# Autodesk Inventor assembly: Montage final
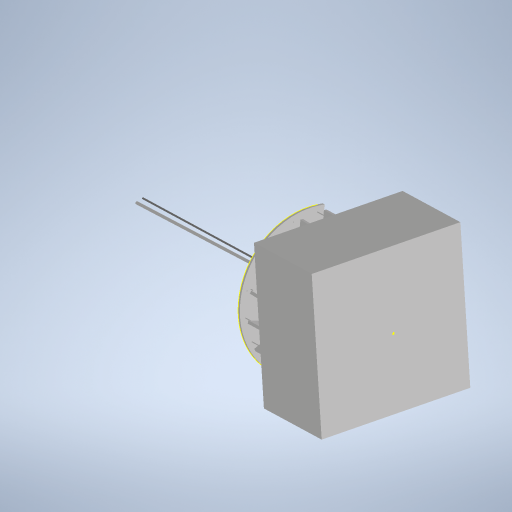
[picture p0: Inventor's stored thumbnail of the model, 512x512]
Saved by Autodesk Inventor 2023 (Build 270158000, 158)
## iProperties
Created: 2022-11-02
Part Number: Montage final
Document SubType Name: Assembly
Designer: Julia
Author: Julia
## Documents named in this file (7)
- C:\Users\Julia\OneDrive\Bureau\PIE\Montage final.iam
- C:\Users\Julia\OneDrive\Bureau\PIE\plaque dessus.ipt
- C:\Users\Julia\OneDrive\Bureau\PIE\plaque de separation.ipt
- C:\Users\Julia\OneDrive\Bureau\PIE\barre plaque.ipt
- C:\Users\Julia\OneDrive\Bureau\PIE\tube acier.ipt
- C:\Users\Julia\OneDrive\Bureau\PIE\tige filetée.ipt
- C:\Users\Julia\OneDrive\Bureau\PIE\bloc percé.ipt
## Components (36 placed, 6 different names)
1. plaque dessus:1 — Rigide:1, Placage:2, Placage:3, Placage:4, Placage:5, Placage:6, Placage:7, Placage:8, Placage:9, Placage:10, Placage:11, Placage:12
2. plaque de separation:1
3. plaque de separation:2 — Placage:8
4. plaque de separation:3 — Placage:11
5. plaque de separation:4 — Placage:10
6. plaque de separation:5 — Placage:9
7. plaque de separation:6 — Placage:3, Logement:6, Logement:19
8. plaque de separation:7 — Placage:5, Logement:7, Logement:8
9. plaque de separation:8 — Placage:6, Logement:12, Logement:13
10. plaque de separation:9 — Placage:12, Logement:3, Logement:4
11. plaque de separation:10 — Placage:7, Logement:20
12. plaque de separation:11 — Placage:4, Logement:1, Logement:2
13. plaque dessus:2 — Placage:13, Logement:14, Logement:15, Logement:16, Placage:14, Placage:15
14. barre plaque:1
15. barre plaque:2
16. barre plaque:3
17. barre plaque:4
18. barre plaque:5
19. barre plaque:6 — Logement:4
20. barre plaque:7
21. barre plaque:8 — Logement:3
22. barre plaque:9
23. barre plaque:10 — Logement:6
24. barre plaque:11 — Logement:2, Logement:16
25. barre plaque:12 — Logement:19, Placage:14
26. barre plaque:13 — Logement:13, Logement:14
27. barre plaque:14 — Logement:20
28. barre plaque:15 — Placage:13
29. barre plaque:16
30. barre plaque:17 — Logement:12
31. barre plaque:18 — Logement:7
32. barre plaque:19 — Logement:8, Placage:15
33. barre plaque:20 — Logement:1, Logement:15
34. tube acier:1
35. tige filetée:1 — Rigide:1, Placage:1
36. bloc percé:1 — Placage:1, Placage:2
## Relationships (30: Mate 15, Insert 14, WeldJoint 1)
- Rigide:1 [WeldJoint] (300 mm): plaque dessus:1 ↔ tige filetée:1
- Placage:1 [Mate]: tige filetée:1 ↔ bloc percé:1
- Placage:2 [Mate]: plaque dessus:1 ↔ bloc percé:1
- Placage:3 [Mate]: plaque dessus:1 ↔ plaque de separation:6
- Placage:4 [Mate]: plaque dessus:1 ↔ plaque de separation:11
- Placage:5 [Mate]: plaque dessus:1 ↔ plaque de separation:7
- Placage:6 [Mate]: plaque dessus:1 ↔ plaque de separation:8
- Placage:7 [Mate]: plaque dessus:1 ↔ plaque de separation:10
- Placage:8 [Mate]: plaque dessus:1 ↔ plaque de separation:2
- Placage:9 [Mate]: plaque dessus:1 ↔ plaque de separation:5
- Placage:10 [Mate]: plaque dessus:1 ↔ plaque de separation:4
- Placage:11 [Mate]: plaque dessus:1 ↔ plaque de separation:3
- Placage:12 [Mate]: plaque dessus:1 ↔ plaque de separation:9
- Placage:13 [Mate] (10 mm): plaque dessus:2 ↔ barre plaque:15
- Logement:1 [Insert]: plaque de separation:11 ↔ barre plaque:20
- Logement:2 [Insert]: plaque de separation:11 ↔ barre plaque:11
- Logement:3 [Insert]: plaque de separation:9 ↔ barre plaque:8
- Logement:4 [Insert]: plaque de separation:9 ↔ barre plaque:6
- Logement:6 [Insert]: plaque de separation:6 ↔ barre plaque:10
- Logement:7 [Insert]: plaque de separation:7 ↔ barre plaque:18
- Logement:8 [Insert]: plaque de separation:7 ↔ barre plaque:19
- Logement:12 [Insert]: plaque de separation:8 ↔ barre plaque:17
- Logement:13 [Insert]: plaque de separation:8 ↔ barre plaque:13
- Logement:14 [Insert]: plaque dessus:2 ↔ barre plaque:13
- Logement:15 [Insert]: plaque dessus:2 ↔ barre plaque:20
- Logement:16 [Insert]: plaque dessus:2 ↔ barre plaque:11
- Logement:19 [Insert]: plaque de separation:6 ↔ barre plaque:12
- Placage:14 [Mate]: plaque dessus:2 ↔ barre plaque:12
- Placage:15 [Mate]: plaque dessus:2 ↔ barre plaque:19
- Logement:20 [Insert]: plaque de separation:10 ↔ barre plaque:14
